# Autodesk Inventor assembly: Assembly Lifting Mechanism
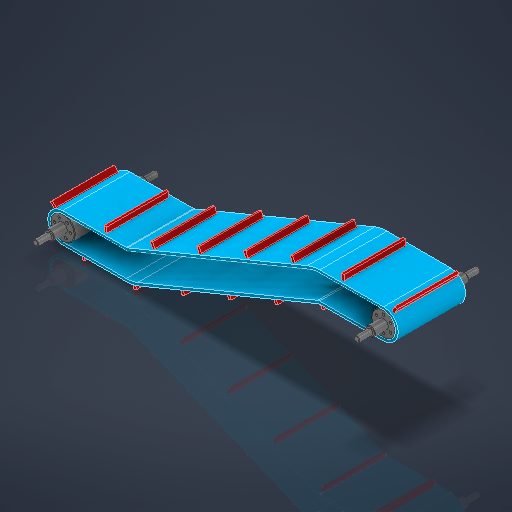
[picture p0: Inventor's stored thumbnail of the model, 512x512]
Saved by Autodesk Inventor 2026.2 (Build 302298010, 298A)
## iProperties
Created: 2026-04-10
Part Number: Assembly Lifting Mechanism
Document SubType Name: Assembly
Designer: yassi
Author: yassi
## Documents named in this file (5)
- C:\Users\yassi\OneDrive\Documents\Inventor\Assembly Lifting Mechanism.iam
- C:\Users\yassi\OneDrive\Documents\Inventor\Part1 Belt before factor.ipt
- C:\Users\yassi\OneDrive\Documents\Inventor\Attatchment.ipt
- C:\Users\yassi\OneDrive\Documents\Inventor\Part1 Belt before factor - Copy BELT.ipt
- C:\Users\yassi\OneDrive\Documents\Inventor\Shaft.ipt
## Components (19 placed, 4 different names)
1. Part1 Belt before factor:1 — Flush:1, Flush:2, Flush:3, Mate:1
2. Part1 Belt before factor - Copy BELT:1 — Flush:4, Flush:5, Flush:6, Mate:2, Mate:3, Flush:7
3. Shaft:1 — Mate:2, Flush:7, Flush:8, Rotation:1
4. Shaft:2 — Mate:3, Flush:8, Rotation:1, Angle:4
5. Attatchment:1 — Mate:1, Angle:1, Angle:2, Angle:3
6. Attatchment:2
7. Attatchment:3
8. Attatchment:4
9. Attatchment:5
10. Attatchment:6
11. Attatchment:7
12. Attatchment:8
13. Attatchment:9
14. Attatchment:10
15. Attatchment:11
16. Attatchment:12
17. Attatchment:13
18. Attatchment:14
19. Attatchment:15
## Component patterns: (15 elements, first: Attatchment:1)
## Relationships (16: Flush 8, Angle 4, Mate 3, RelateRotation 1)
- Flush:1: Part1 Belt before factor:1
- Flush:2: Part1 Belt before factor:1
- Flush:3: Part1 Belt before factor:1
- Mate:1: Part1 Belt before factor:1 ↔ Attatchment:1
- Angle:1 (0 deg): Attatchment:1
- Angle:2 (0 deg): Attatchment:1
- Angle:3 (0 deg): Attatchment:1
- Flush:4: Part1 Belt before factor - Copy BELT:1
- Flush:5: Part1 Belt before factor - Copy BELT:1
- Flush:6: Part1 Belt before factor - Copy BELT:1
- Mate:2: Part1 Belt before factor - Copy BELT:1 ↔ Shaft:1
- Mate:3: Part1 Belt before factor - Copy BELT:1 ↔ Shaft:2
- Flush:7: Part1 Belt before factor - Copy BELT:1 ↔ Shaft:1
- Flush:8: Shaft:1 ↔ Shaft:2
- Rotation:1 [RelateRotation] (1 ul): Shaft:1 ↔ Shaft:2
- Angle:4 (0 deg): Shaft:2
